# Autodesk Inventor assembly: Very Basic JOint
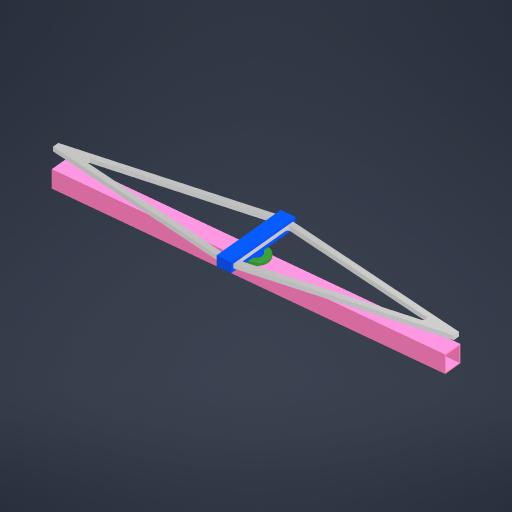
[picture p0: Inventor's stored thumbnail of the model, 512x512]
Saved by Autodesk Inventor 2023 (Build 270158000, 158)
## iProperties
Created: 2023-03-16
Part Number: Very Basic JOint
Document SubType Name: Assembly
Designer: bugme
Author: bugme
## Documents named in this file (6)
- C:\Users\bugme\Desktop\Diff Bar\Very Basic JOint.iam
- C:\Users\bugme\Desktop\Diff Bar\Main Support.ipt
- C:\Users\bugme\Documents\GitHub\BehrendURCMechanical\CAD\Chassis V3\aluminumextrusiontool.ipt
- C:\Users\bugme\Documents\GitHub\BehrendURCMechanical\CAD\Chassis V3\aluminumextrusiontool\aluminumextrusiontool-54.ipt
- C:\Users\bugme\Desktop\Diff Bar\Bracket.ipt
- C:\Users\bugme\Downloads\6384K363_Ball Bearing.ipt
## Components (4 placed, 4 different names)
1. Main Support:1 — Rigid:1
2. aluminumextrusiontool-54:2 — Cylindrical:1, Angle:1
3. Bracket:1 — Rigid:1, Cylindrical:1, Angle:1, Cylindrical:2
4. 6384K363_Ball Bearing:1 — Cylindrical:2
## Relationships (4: CylindricalJoint 2, WeldJoint 1, Angle 1)
- Rigid:1 [WeldJoint]: Main Support:1 ↔ Bracket:1
- Cylindrical:1: aluminumextrusiontool-54:2 ↔ Bracket:1
- Angle:1 (90 deg): aluminumextrusiontool-54:2 ↔ Bracket:1
- Cylindrical:2: Bracket:1 ↔ 6384K363_Ball Bearing:1
